# Autodesk Inventor assembly: Beginning_assembly
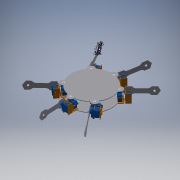
[picture p0: Inventor's stored thumbnail of the model, 180x180]
Saved by Autodesk Inventor 2016 (Build 200138000, 138)
## iProperties
Created: 2015-10-08
Part Number: Beginning_assembly
Document SubType Name: Assembly
Designer: powasar16
Author: powasar16
## Documents named in this file (8)
- C:\Users\powasar16\Documents\GitHub\SpyderRobot\Inventor\Created Parts\Beginning_assembly.iam
- C:\Users\powasar16\Documents\GitHub\SpyderRobot\Inventor\Created Parts\Arduino.ipt
- C:\Users\powasar16\Documents\GitHub\SpyderRobot\Inventor\Created Parts\Base_bottom.ipt
- C:\Users\powasar16\Documents\GitHub\SpyderRobot\Inventor\Imported Parts\Motherboard Standoff 12mm M3x0.5.ipt
- C:\Users\powasar16\Documents\GitHub\SpyderRobot\Inventor\Created Parts\Servo_vice.ipt
- C:\Users\powasar16\Documents\GitHub\SpyderRobot\Inventor\Created Parts\Servo.iam
- C:\Users\powasar16\Documents\GitHub\SpyderRobot\Inventor\Created Parts\Leg.ipt
- C:\Users\powasar16\Documents\GitHub\SpyderRobot\Inventor\Created Parts\Toe.ipt
## Components (42 placed, 7 different names)
1. Arduino:1 — Mate:2, Mate:3, Mate:4, Mate:5, Mate:14, Mate:15, Mate:16, Mate:17, Mate:18, Mate:19, Mate:20, Mate:21, Mate:22
2. Base_bottom:1 — Mate:2, Mate:3, Mate:4, Mate:5, Mate:6, Mate:7, Mate:8, Mate:9, Mate:10, Mate:11, Mate:12, Mate:13, Mate:29, Mate:80, Mate:81
3. Motherboard Standoff 12mm M3x0.5:1 — Mate:7, Mate:12
4. Motherboard Standoff 12mm M3x0.5:2 — Mate:6, Mate:11, Mate:14
5. Motherboard Standoff 12mm M3x0.5:3 — Mate:9, Mate:13
6. Motherboard Standoff 12mm M3x0.5:4 — Mate:8, Mate:10
7. Motherboard Standoff 12mm M3x0.5:5 — Mate:15, Mate:16
8. Motherboard Standoff 12mm M3x0.5:6 — Mate:21, Mate:22
9. Motherboard Standoff 12mm M3x0.5:7 — Mate:19, Mate:20
10. Motherboard Standoff 12mm M3x0.5:8 — Mate:17, Mate:18
11. Base_bottom:2 — Flush:1, Flush:2, Flush:3, Flush:4, Flush:5, Mate:48, Flush:6, Mate:80, Mate:81, Mate:82, Mate:83, Mate:84, Mate:85, Mate:86, Angle:1, Angle:2, Angle:3, Angle:4, Angle:5, Angle:6
12. Servo_vice:1 — Mate:25, Mate:26, Mate:27, Mate:29, Mate:63, Mate:64
13. Servo:1 [sub-assembly] — Mate:25, Mate:26, Mate:27, Flush:1, Mate:86
14. Servo_vice:2 — Mate:61, Mate:62
15. Servo:2 [sub-assembly] — Flush:2, Mate:85
16. Servo_vice:3 — Mate:53, Mate:54
17. Servo:3 [sub-assembly] — Flush:3, Mate:84
18. Servo:4 [sub-assembly] — Mate:38, Mate:39, Mate:40, Flush:4, Mate:83
19. Servo_vice:4 — Mate:38, Mate:39, Mate:40, Mate:78, Mate:79
20. Servo:5 [sub-assembly] — Flush:5, Mate:82
21. Servo_vice:5 — Mate:76, Mate:77
22. Servo:6 [sub-assembly] — Mate:48, Flush:6
23. Servo_vice:6 — Mate:74, Mate:75
24. Servo_vice:7 — Mate:53, Mate:54
25. Servo:7 [sub-assembly] — Angle:3, Mate:90, Mate:91
26. Servo_vice:8 — Mate:61, Mate:62
27. Servo:8 [sub-assembly] — Angle:2, Mate:88, Mate:89
28. Servo_vice:9 — Mate:63, Mate:64
29. Servo:9 [sub-assembly] — Angle:1, Mate:87
30. Servo:10 [sub-assembly] — Angle:6, Mate:96, Mate:97
31. Servo_vice:10 — Mate:74, Mate:75
32. Servo:11 [sub-assembly] — Angle:5, Mate:94, Mate:95
33. Servo_vice:11 — Mate:76, Mate:77
34. Servo:12 [sub-assembly] — Angle:4, Mate:92, Mate:93
35. Servo_vice:12 — Mate:78, Mate:79
36. Leg:1 — Mate:87
37. Leg:2 — Mate:88, Mate:89
38. Leg:3 — Mate:90, Mate:91
39. Leg:4 — Mate:92, Mate:93
40. Leg:5 — Mate:94, Mate:95
41. Leg:6 — Mate:96, Mate:97
42. Toe:1
## Relationships (101: Mate 89, Flush 6, Angle 6)
- Mate:2: Arduino:1 ↔ Base_bottom:1
- Mate:3: Arduino:1 ↔ Base_bottom:1
- Mate:4: Arduino:1 ↔ Base_bottom:1
- Mate:5: Arduino:1 ↔ Base_bottom:1
- Mate:6: Base_bottom:1 ↔ Motherboard Standoff 12mm M3x0.5:2
- Mate:7: Base_bottom:1 ↔ Motherboard Standoff 12mm M3x0.5:1
- Mate:8: Base_bottom:1 ↔ Motherboard Standoff 12mm M3x0.5:4
- Mate:9: Base_bottom:1 ↔ Motherboard Standoff 12mm M3x0.5:3
- Mate:10: Base_bottom:1 ↔ Motherboard Standoff 12mm M3x0.5:4
- Mate:11: Base_bottom:1 ↔ Motherboard Standoff 12mm M3x0.5:2
- Mate:12: Base_bottom:1 ↔ Motherboard Standoff 12mm M3x0.5:1
- Mate:13: Base_bottom:1 ↔ Motherboard Standoff 12mm M3x0.5:3
- Mate:14: Arduino:1 ↔ Motherboard Standoff 12mm M3x0.5:2
- Mate:15: Arduino:1 ↔ Motherboard Standoff 12mm M3x0.5:5
- Mate:16: Arduino:1 ↔ Motherboard Standoff 12mm M3x0.5:5
- Mate:17: Arduino:1 ↔ Motherboard Standoff 12mm M3x0.5:8
- Mate:18: Arduino:1 ↔ Motherboard Standoff 12mm M3x0.5:8
- Mate:19: Arduino:1 ↔ Motherboard Standoff 12mm M3x0.5:7
- Mate:20: Arduino:1 ↔ Motherboard Standoff 12mm M3x0.5:7
- Mate:21: Arduino:1 ↔ Motherboard Standoff 12mm M3x0.5:6
- Mate:22: Arduino:1 ↔ Motherboard Standoff 12mm M3x0.5:6
- Mate:25: Servo_vice:1 ↔ Servo:1
- Mate:26: Servo_vice:1 ↔ Servo:1
- Mate:27: Servo_vice:1 ↔ Servo:1
- Mate:29 (1.905 mm): Base_bottom:1 ↔ Servo_vice:1
- Flush:1: Base_bottom:2 ↔ Servo:1
- [Mate]: Servo_vice:2 ↔ Servo:2
- [Mate]: Servo_vice:2 ↔ Servo:2
- [Mate]: Servo_vice:2 ↔ Servo:2
- [Mate]: Servo_vice:3 ↔ Servo:3
- [Mate]: Servo_vice:3 ↔ Servo:3
- [Mate]: Servo_vice:3 ↔ Servo:3
- Flush:2: Base_bottom:2 ↔ Servo:2
- Flush:3: Base_bottom:2 ↔ Servo:3
- Mate:38: Servo:4 ↔ Servo_vice:4
- Mate:39: Servo:4 ↔ Servo_vice:4
- Mate:40: Servo:4 ↔ Servo_vice:4
- [Mate]: Servo:5 ↔ Servo_vice:5
- [Mate]: Servo:5 ↔ Servo_vice:5
- [Mate]: Servo:5 ↔ Servo_vice:5
- [Mate]: Servo:6 ↔ Servo_vice:6
- [Mate]: Servo:6 ↔ Servo_vice:6
- [Mate]: Servo:6 ↔ Servo_vice:6
- Flush:4: Base_bottom:2 ↔ Servo:4
- Flush:5: Base_bottom:2 ↔ Servo:5
- Mate:48: Base_bottom:2 ↔ Servo:6
- Flush:6: Base_bottom:2 ↔ Servo:6
- [Mate]: Servo_vice:7 ↔ Servo:7
- [Mate]: Servo_vice:7 ↔ Servo:7
- [Mate]: Servo_vice:7 ↔ Servo:7
- Mate:53 (3.175 mm): Servo_vice:3 ↔ Servo_vice:7
- Mate:54: Servo_vice:3 ↔ Servo_vice:7
- [Mate]: Servo_vice:8 ↔ Servo:8
- [Mate]: Servo_vice:8 ↔ Servo:8
- [Mate]: Servo_vice:8 ↔ Servo:8
- [Mate]: Servo_vice:9 ↔ Servo:9
- [Mate]: Servo_vice:9 ↔ Servo:9
- [Mate]: Servo_vice:9 ↔ Servo:9
- Mate:61: Servo_vice:2 ↔ Servo_vice:8
- Mate:62 (3.175 mm): Servo_vice:2 ↔ Servo_vice:8
- Mate:63: Servo_vice:1 ↔ Servo_vice:9
- Mate:64 (3.175 mm): Servo_vice:1 ↔ Servo_vice:9
- [Mate]: Servo:10 ↔ Servo_vice:10
- [Mate]: Servo:10 ↔ Servo_vice:10
- [Mate]: Servo:10 ↔ Servo_vice:10
- [Mate]: Servo:11 ↔ Servo_vice:11
- [Mate]: Servo:11 ↔ Servo_vice:11
- [Mate]: Servo:11 ↔ Servo_vice:11
- [Mate]: Servo:12 ↔ Servo_vice:12
- [Mate]: Servo:12 ↔ Servo_vice:12
- [Mate]: Servo:12 ↔ Servo_vice:12
- Mate:74: Servo_vice:6 ↔ Servo_vice:10
- Mate:75 (3.175 mm): Servo_vice:6 ↔ Servo_vice:10
- Mate:76: Servo_vice:5 ↔ Servo_vice:11
- Mate:77 (3.175 mm): Servo_vice:5 ↔ Servo_vice:11
- Mate:78: Servo_vice:4 ↔ Servo_vice:12
- Mate:79 (3.175 mm): Servo_vice:4 ↔ Servo_vice:12
- Mate:80: Base_bottom:1 ↔ Base_bottom:2
- Mate:81: Base_bottom:1 ↔ Base_bottom:2
- Mate:82: Base_bottom:2 ↔ Servo:5
- Mate:83: Base_bottom:2 ↔ Servo:4
- Mate:84: Base_bottom:2 ↔ Servo:3
- Mate:85: Base_bottom:2 ↔ Servo:2
- Mate:86: Base_bottom:2 ↔ Servo:1
- Angle:1 (0 deg): Base_bottom:2 ↔ Servo:9
- Mate:87: Servo:9 ↔ Leg:1
- Angle:2 (0 deg): Base_bottom:2 ↔ Servo:8
- Angle:3 (0 deg): Base_bottom:2 ↔ Servo:7
- Angle:4 (0 deg): Base_bottom:2 ↔ Servo:12
- Angle:5 (0 deg): Base_bottom:2 ↔ Servo:11
- Angle:6 (0 deg): Base_bottom:2 ↔ Servo:10
- Mate:88: Servo:8 ↔ Leg:2
- Mate:89: Servo:8 ↔ Leg:2
- Mate:90: Servo:7 ↔ Leg:3
- Mate:91: Servo:7 ↔ Leg:3
- Mate:92: Servo:12 ↔ Leg:4
- Mate:93: Servo:12 ↔ Leg:4
- Mate:94: Servo:11 ↔ Leg:5
- Mate:95: Servo:11 ↔ Leg:5
- Mate:96: Servo:10 ↔ Leg:6
- Mate:97: Servo:10 ↔ Leg:6
## Named parameters: d32_d26 = 0 mm, d33_d27 = 0 mm, d34_d28 = 0 mm, d35_d26 = 0 mm, d36_d27 = 0 mm, d37_d28 = 0 mm, d45_d42 = 0 mm, d46_d43 = 0 mm, d47_d44 = 0 mm, d48_d42 = 0 mm, d49_d43 = 0 mm, d50_d44 = 0 mm, d57_d26 = 0 mm, d58_d27 = 0 mm, d59_d28 = 0 mm, d63_d57_d26 = 0 mm, d64_d58_d27 = 0 mm, d65_d59_d28 = 0 mm, d66_d63_d57_d26 = 0 mm, d67_d64_d58_d27 = 0 mm, d68_d65_d59_d28 = 0 mm, d73_d48_d42 = 0 mm, d74_d49_d43 = 0 mm, d75_d50_d44 = 0 mm, d76_d73_d48_d42 = 0 mm, d77_d74_d49_d43 = 0 mm, d78_d75_d50_d44 = 0 mm, d79_d73_d48_d42 = 0 mm, d80_d74_d49_d43 = 0 mm, d81_d75_d50_d44 = 0 mm
